# Autodesk Inventor assembly: 下半身_6
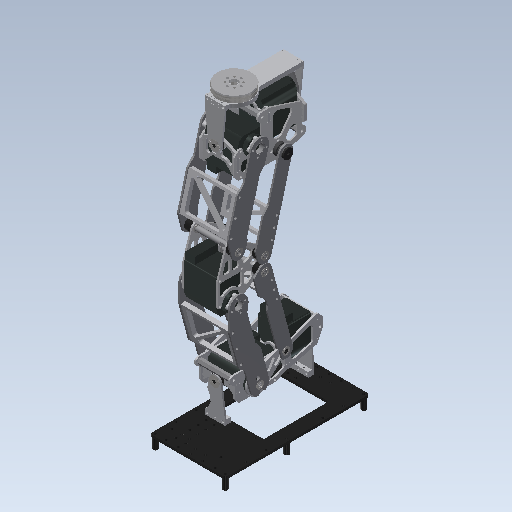
[picture p0: Inventor's stored thumbnail of the model, 512x512]
Saved by Autodesk Inventor 2020 (Build 240168000, 168)
## iProperties
Created: 2016-08-23
Part Number: 下半身_6
Material: 一般
Document SubType Name: Assembly
Designer: hiro
Mass: 983.506 g
Surface Area: 2507.77 cm^2
Volume: 440.119 cm^3
Density: 2.23464 g/cm^3
Author: hiro
## Documents named in this file (15)
- C:\Users\hiroki\Documents\OpenPlatform_ver3_0\下半身_6.iam
- C:\Users\hiroki\Documents\OpenPlatform_ver3_0\下半身_160823\膝\膝_6_1.iam
- C:\Users\hiroki\Documents\OpenPlatform_ver3_0\下半身\足首\足首_1.iam
- C:\Users\hiroki\Documents\OpenPlatform_ver3_0\下半身\足首\足首_独立ピッチ_1.iam
- C:\Users\hiroki\Documents\OpenPlatform_ver3_0\下半身_160823\リンク\リンク_6_2.iam
- C:\Users\hiroki\Documents\OpenPlatform_ver3_0\下半身\足裏\足裏_1_1.iam
- C:\Users\hiroki\Documents\OpenPlatform_ver3_0\下半身_160823\リンク\リンク_6_3.iam
- C:\Users\hiroki\Documents\OpenPlatform_ver3_0\下半身_160823\リンク\リンク_6_4.iam
- C:\Users\hiroki\Documents\OpenPlatform_ver3_0\下半身_160823\付け根\付け根_1.iam
- C:\Users\hiroki\Documents\OpenPlatform_ver3_0\下半身_160823\付け根ロール\付け根ロール_1.iam
- C:\Users\hiroki\Documents\OpenPlatform_ver3_0\下半身_160823\付け根ロール\長穴減速_ホーン_2_1.iam
- C:\Users\hiroki\Documents\OpenPlatform_ver3_0\下半身_160823\リンク\長穴減速_ホーン_2_2.iam
- C:\Users\hiroki\Documents\OpenPlatform_ver3_0\下半身_160823\リンク\リンク_ふくらはぎ_サブフレーム_1_4.ipt
- C:\Users\hiroki\Documents\OpenPlatform_ver3_0\下半身_160823\リンク\リンク_6_1.iam
- C:\Users\hiroki\Documents\OpenPlatform_ver3_0\既製品\WSSS12-10-6.ipt
## Components (20 placed, 14 different names)
1. 付け根ロール_1:1 [sub-assembly] — 角度:10, 角度:22, メイト:23, フラッシュ:25, フラッシュ:26, 角度:3, メイト:28, 挿入:85
2. 膝_6_1:1 [sub-assembly] — 挿入:58, 挿入:59, 挿入:64, 角度:30, 挿入:77, 挿入:78, 角度:33, 挿入:89, 挿入:90
3. 足首_1:1 [sub-assembly] — 挿入:12, 挿入:22, 角度:31, 挿入:81
4. 足首_独立ピッチ_1:1 [sub-assembly] — 挿入:22, 挿入:81, 挿入:84, 挿入:87
5. 足裏_1_1:1 [sub-assembly] — 挿入:12, 角度:3
6. 付け根_1:1 [sub-assembly] — 挿入:18, 角度:10, 角度:22, 挿入:50, 挿入:51, 挿入:74, 挿入:75, 角度:30, 角度:31, 角度:32, 挿入:85, 挿入:91
7. 長穴減速_ホーン_2_1:1 [sub-assembly] — 挿入:18, メイト:28, 挿入:88
8. リンク_6_3:1 [sub-assembly] — 挿入:64, 挿入:91
9. リンク_6_4:1 [sub-assembly] — 挿入:68, 角度:32, 挿入:89, 挿入:92, 挿入:94
10. 長穴減速_ホーン_2_2:2 [sub-assembly] — 挿入:88
11. リンク_ふくらはぎ_サブフレーム_1_4:1 — 挿入:50, 挿入:51, 挿入:68
12. リンク_ふくらはぎ_サブフレーム_1_4:2 — 挿入:74, 挿入:75
13. リンク_ふくらはぎ_サブフレーム_1_4:3 — 挿入:58, 挿入:59, 挿入:83
14. リンク_ふくらはぎ_サブフレーム_1_4:4 — 挿入:77, 挿入:78
15. リンク_6_2:2 [sub-assembly] — 挿入:83, 挿入:84, 角度:33, 挿入:93, 挿入:95
16. リンク_6_1:1 [sub-assembly] — 挿入:87, 挿入:90
17. WSSS12-10-6:1 — 挿入:95
18. WSSS12-10-6:2 — 挿入:92
19. WSSS12-10-6:3 — 挿入:93
20. WSSS12-10-6:4 — 挿入:94
## Relationships (37: Insert 26, Angle 7, Mate 2, Flush 2)
- 挿入:12 [Insert]: 足首_1:1 ↔ 足裏_1_1:1
- 角度:3 [Angle] (180 deg): 付け根ロール_1:1 ↔ 足裏_1_1:1
- 挿入:18 [Insert]: 付け根_1:1 ↔ 長穴減速_ホーン_2_1:1
- 角度:10 [Angle] (-45 deg): 付け根ロール_1:1 ↔ 付け根_1:1
- 角度:22 [Angle] (20 deg): 付け根ロール_1:1 ↔ 付け根_1:1
- メイト:23 [Mate]: 付け根ロール_1:1
- フラッシュ:25 [Flush]: 付け根ロール_1:1
- フラッシュ:26 [Flush]: 付け根ロール_1:1
- 挿入:22 [Insert]: 足首_1:1 ↔ 足首_独立ピッチ_1:1
- 挿入:50 [Insert]: 付け根_1:1 ↔ リンク_ふくらはぎ_サブフレーム_1_4:1
- 挿入:51 [Insert]: 付け根_1:1 ↔ リンク_ふくらはぎ_サブフレーム_1_4:1
- メイト:28 [Mate]: 付け根ロール_1:1 ↔ 長穴減速_ホーン_2_1:1
- 挿入:58 [Insert]: 膝_6_1:1 ↔ リンク_ふくらはぎ_サブフレーム_1_4:3
- 挿入:59 [Insert]: 膝_6_1:1 ↔ リンク_ふくらはぎ_サブフレーム_1_4:3
- 挿入:64 [Insert]: 膝_6_1:1 ↔ リンク_6_3:1
- 挿入:68 [Insert]: リンク_6_4:1 ↔ リンク_ふくらはぎ_サブフレーム_1_4:1
- 挿入:74 [Insert]: 付け根_1:1 ↔ リンク_ふくらはぎ_サブフレーム_1_4:2
- 挿入:75 [Insert]: 付け根_1:1 ↔ リンク_ふくらはぎ_サブフレーム_1_4:2
- 角度:30 [Angle] (0 deg): 膝_6_1:1 ↔ 付け根_1:1
- 角度:31 [Angle] (0 deg): 足首_1:1 ↔ 付け根_1:1
- 挿入:77 [Insert]: 膝_6_1:1 ↔ リンク_ふくらはぎ_サブフレーム_1_4:4
- 挿入:78 [Insert]: 膝_6_1:1 ↔ リンク_ふくらはぎ_サブフレーム_1_4:4
- 挿入:81 [Insert]: 足首_1:1 ↔ 足首_独立ピッチ_1:1
- 挿入:83 [Insert]: リンク_ふくらはぎ_サブフレーム_1_4:3 ↔ リンク_6_2:2
- 挿入:84 [Insert]: 足首_独立ピッチ_1:1 ↔ リンク_6_2:2
- 角度:32 [Angle] (15 deg): 付け根_1:1 ↔ リンク_6_4:1
- 挿入:85 [Insert]: 付け根ロール_1:1 ↔ 付け根_1:1
- 角度:33 [Angle] (-15 deg): 膝_6_1:1 ↔ リンク_6_2:2
- 挿入:87 [Insert]: 足首_独立ピッチ_1:1 ↔ リンク_6_1:1
- 挿入:88 [Insert]: 長穴減速_ホーン_2_1:1 ↔ 長穴減速_ホーン_2_2:2
- 挿入:89 [Insert]: 膝_6_1:1 ↔ リンク_6_4:1
- 挿入:90 [Insert]: 膝_6_1:1 ↔ リンク_6_1:1
- 挿入:91 [Insert]: 付け根_1:1 ↔ リンク_6_3:1
- 挿入:92 [Insert]: リンク_6_4:1 ↔ WSSS12-10-6:2
- 挿入:93 [Insert]: リンク_6_2:2 ↔ WSSS12-10-6:3
- 挿入:94 [Insert]: リンク_6_4:1 ↔ WSSS12-10-6:4
- 挿入:95 [Insert]: リンク_6_2:2 ↔ WSSS12-10-6:1
